# Autodesk Inventor assembly: каретка
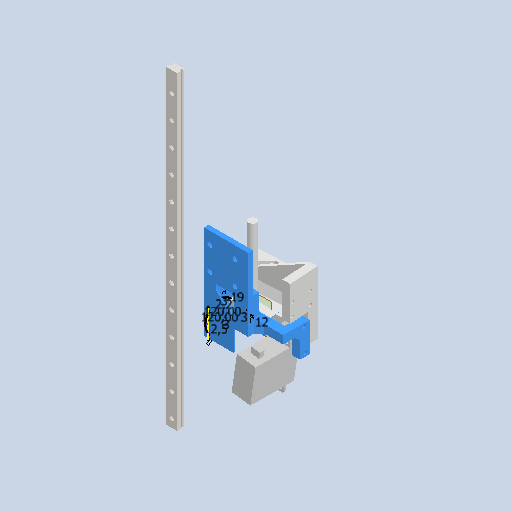
[picture p0: Inventor's stored thumbnail of the model, 512x512]
Saved by Autodesk Inventor 2024.2 (Build 282272000, 272)
## iProperties
Created: 2026-01-30
Part Number: каретка
Document SubType Name: Assembly
Designer: Service
Author: Service
## Documents named in this file (7)
- C:\Users\Service\Documents\Artist-v2\3D\каретка.iam
- C:\Users\Service\Documents\Artist-v2\3D\крепежная основа.ipt
- C:\Users\Service\Documents\Artist\3D\стл\Сборка плоттер\Сервопривод.ipt
- C:\Users\Service\Documents\Artist\3D\стл\Сборка плоттер\Деталь.ipt
- C:\Users\Service\Documents\Artist-v2\3D\stl\вал с пружиной.ipt
- C:\Users\Service\Documents\Artist-v2\3D\stl\каретка.ipt
- C:\Users\Service\Documents\Artist-v2\3D\MGN7.ipt
## Components (6 placed, 6 different names)
1. крепежная основа:1 — Заподлицо:1, Совмещение:7, Совмещение:9, Совмещение:11
2. Сервопривод:1 — Совмещение:9, Совмещение:10, Совмещение:11, Совмещение:12
3. Деталь:1 — Совмещение:10, Совмещение:12
4. вал с пружиной:1 — Совмещение:7, Совмещение:13
5. каретка:1 — Заподлицо:1, Совмещение:13
6. MGN7:1
## Relationships (7: Mate 6, Flush 1)
- Заподлицо:1 [Flush]: крепежная основа:1 ↔ каретка:1
- Совмещение:7 [Mate]: крепежная основа:1 ↔ вал с пружиной:1
- Совмещение:9 [Mate]: крепежная основа:1 ↔ Сервопривод:1
- Совмещение:10 [Mate]: Сервопривод:1 ↔ Деталь:1
- Совмещение:11 [Mate]: крепежная основа:1 ↔ Сервопривод:1
- Совмещение:12 [Mate]: Сервопривод:1 ↔ Деталь:1
- Совмещение:13 [Mate]: вал с пружиной:1 ↔ каретка:1
